# Autodesk Inventor assembly: Stand Assembly Roll 44
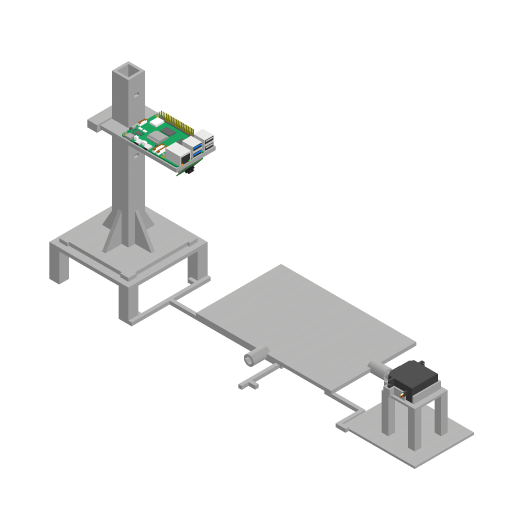
[picture p0: Inventor's stored thumbnail of the model, 512x512]
Saved by Autodesk Inventor 2023.4 (Build 274418000, 418)
## iProperties
Created: 2024-02-27
Part Number: Stand Assembly Roll 44
Document SubType Name: Assembly
Designer: josep
Author: josep
## iProperties of the stored document pitchrollmount44.ipt
Created: 2024-03-15
Part Number: pitchrollmount44
Material: Generic
Document SubType Name: Modeling
Designer: josep
Density: 1 g/cm^3
Appearance: Default
Sending System: Autodesk Inventor 2024
__%SI_4: josep
__%DT_4: 2024-03-15
__%DT_5: pitchrollmount44
__%DT_11: 1970-01-01
__%DT_13: 1970-01-01
__%DT_20: Generic
__%DT_32: Modeling
__%DT_33: 1970-01-01
__%DT_35: 1970-01-01
__%DT_40: 1
__%DT_41: josep
__%DT_44: False
__%DT_51: False
__%DT_58: 0.0
__%DT_59: 0.0
__%DT_60: 0.0
__%DT_61: 1.0
__%DT_62: 17
__%DT_63: 0.0
__%DT_64: 0.0
__%DT_65: 0.0
__%DT_67: 2024 (Build 280153020, 153B)
__%DT_71: C:\Users\Public\Documents\Autodesk\Inventor 2015\Design Data\Materials\InventorMaterialLibrary.adsklib#1:Generic #MaterialInv_072
__%DT_72: Default
__%DT_73: False
__%DC_6: 1970-01-01
__%DC_8: 1970-01-01
__%DC_13: 7
__%DC_14: 6
__%DC_15: 5
__%DC_16: js3368
__%DC_17: 2024-03-20
Author: josep
## iProperties of the stored document SER0044.ipt
Company: Unknown
Created: 2024-02-13
Part Number: SER0044
Material: Generic
Description: Unknown
Document SubType Name: Modeling
Designer: josep
Authority: Unknown
Density: 1 g/cm^3
Appearance: Default
Sending System: Solid Edge
Preprocessor: ST-DEVELOPER v18.102
Title: SER0044
Author: Unknown
## Documents named in this file (14)
- **C:\Users\josep\OneDrive - University of Bath\Documents\University\Year IV\FYP Ideas\Precision Landing\Bench Test\Stand Assembly Roll 44.iam*LocalDocs*xAaaaa1caAaaaaaaaAaaaqwlyEg*pitchrollmount44.ipt
- **C:\Users\josep\OneDrive - University of Bath\Documents\University\Year IV\FYP Ideas\Precision Landing\Bench Test\Stand Assembly Roll 44.iam*LocalDocs*xAaaaaoaaAaaaaaaaAaaaq1f25d*SER0044.ipt
- C:\Users\josep\OneDrive - University of Bath\Documents\University\Year IV\FYP Ideas\Precision Landing\Bench Test\Stand Assembly Roll 44.iam
- C:\Users\josep\OneDrive - University of Bath\Documents\University\Year IV\FYP Ideas\Precision Landing\Bench Test\Fixture.ipt
- C:\Users\josep\OneDrive - University of Bath\Documents\University\Year IV\FYP Ideas\Precision Landing\Bench Test\Platform.ipt
- C:\Users\josep\OneDrive - University of Bath\Documents\University\Year IV\FYP Ideas\Precision Landing\Bench Test\Stand.ipt
- C:\Users\josep\OneDrive - University of Bath\Documents\University\Year IV\FYP Ideas\Precision Landing\Bench Test\GroundCorrected.ipt
- C:\Users\josep\OneDrive - University of Bath\Documents\University\Year IV\FYP Ideas\Precision Landing\Bench Test\Servo Adapter.ipt
- C:\Users\josep\Downloads\raspberry-pi-5-sbc-1.snapshot.2\raspberry-pi-5-sbc-simple\raspberry-pi-5-sbc-simple.ipt
- C:\Users\josep\Downloads\Raspberry Pi  Camera\Raspberry Pi  Camera.ipt
- C:\Users\josep\OneDrive - University of Bath\Documents\University\Year IV\FYP Ideas\Precision Landing\Bench Test\Stand Legs.ipt
- C:\Users\josep\OneDrive - University of Bath\Documents\University\Year IV\FYP Ideas\Precision Landing\Bench Test\Positioning Stencil.ipt
- C:\Users\josep\Downloads\LIB_SER0044\SER0044\3D\SER0044.stp
- C:\Users\josep\OneDrive - University of Bath\Documents\University\Year IV\FYP Ideas\Precision Landing\Bench Test\pitchrollmount44.ipt
## Components (11 placed, 11 different names)
1. Fixture:1 — Mate:4, Mate:5, Mate:6
2. Platform:1 — Mate:1, Mate:2, Mate:3, Mate:5, Mate:6, Rotational:2, Mate:11, Rotational:3, Mate:12, Mate:13
3. Stand:1 — Mate:1, Mate:2, Mate:3, Mate:4, Mate:14, Flush:3, Flush:4
4. GroundCorrected:1 — Mate:15, Flush:2, Rotational:4
5. Servo Adapter:1 — Rotational:4, Insert:1
6. raspberry-pi-5-sbc-simple:1 — Mate:12, Mate:13
7. Raspberry Pi  Camera:1 — Rotational:2, Mate:11, Rotational:3
8. Stand Legs:1 — Mate:14, Mate:15, Flush:2, Flush:3, Flush:4, Mate:16, Mate:17, Mate:24
9. pitchrollmount44:1 — Mate:18, Mate:19, Mate:20, Mate:21, Mate:23
10. SER0044:1 — Mate:19, Mate:20, Mate:21, Insert:1
11. Positioning Stencil:1 — Mate:22, Mate:23, Mate:24
## Relationships (27: Mate 20, RevoluteJoint 3, Flush 3, Insert 1)
- Mate:1: Platform:1 ↔ Stand:1
- Mate:2: Platform:1 ↔ Stand:1
- Mate:3: Platform:1 ↔ Stand:1
- Mate:4: Fixture:1 ↔ Stand:1
- Mate:5: Fixture:1 ↔ Platform:1
- Mate:6: Fixture:1 ↔ Platform:1
- Rotational:2 [RevoluteJoint]: Platform:1 ↔ Raspberry Pi  Camera:1
- Mate:11: Platform:1 ↔ Raspberry Pi  Camera:1
- Rotational:3 [RevoluteJoint]: Platform:1 ↔ Raspberry Pi  Camera:1
- Mate:12: Platform:1 ↔ raspberry-pi-5-sbc-simple:1
- Mate:13: Platform:1 ↔ raspberry-pi-5-sbc-simple:1
- Mate:14: Stand:1 ↔ Stand Legs:1
- Mate:15 (107.107 mm): GroundCorrected:1 ↔ Stand Legs:1
- Flush:2 (4.5 mm): GroundCorrected:1 ↔ Stand Legs:1
- Flush:3 (10 mm): Stand:1 ↔ Stand Legs:1
- Flush:4 (10 mm): Stand:1 ↔ Stand Legs:1
- Mate:16: Stand Legs:1
- Mate:17: Stand Legs:1
- Rotational:4 [RevoluteJoint]: GroundCorrected:1 ↔ Servo Adapter:1
- Mate:18: pitchrollmount44:1
- Mate:19: pitchrollmount44:1 ↔ SER0044:1
- Mate:20: pitchrollmount44:1 ↔ SER0044:1
- Mate:21: pitchrollmount44:1 ↔ SER0044:1
- Insert:1: Servo Adapter:1 ↔ SER0044:1
- Mate:22: Positioning Stencil:1
- Mate:23: pitchrollmount44:1 ↔ Positioning Stencil:1
- Mate:24: Stand Legs:1 ↔ Positioning Stencil:1
